# Autodesk Inventor assembly: drivebay
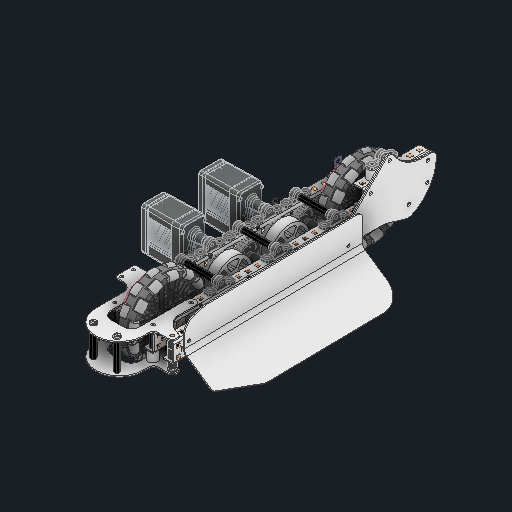
[picture p0: Inventor's stored thumbnail of the model, 512x512]
Saved by Autodesk Inventor 2024 (Build 280153000, 153)
## iProperties
Created: 2023-08-15
Part Number: drivebay
Document SubType Name: Assembly
Designer: avere
Author: avere
## Documents named in this file (25)
- D:\vex_robotics\hardware\cad\spades_v0.1\chassis\drivebay.iam
- D:\vex_robotics\hardware\cad\spades_v0.1\chassis\outer.iam
- D:\vex_robotics\hardware\cad\spades_v0.1\chassis\inner.iam
- D:\vex_robotics\hardware\cad\spades_v0.1\chassis\wheel.iam
- D:\vex_robotics\hardware\cad\spades_v0.1\chassis\gear.iam
- D:\vex_robotics\hardware\cad\VEX-CAD-Inventor-1.41\Motion\Spacers\Spacer Nylon .500 OD\NSpacer White .500 OD x .500.ipt
- D:\vex_robotics\hardware\cad\spades_v0.1\chassis\custom_parts\gusset.ipt
- D:\vex_robotics\hardware\cad\VEX-CAD-Inventor-1.41\Structure\Standoff\Standoff 1.50.ipt
- D:\vex_robotics\hardware\cad\VEX-CAD-Inventor-1.41\Motion\Spacers\Spacer Nylon .375 OD\NSpacer .375 OD x .125.ipt
- D:\vex_robotics\hardware\cad\spades_v0.1\chassis\flapper.iam
- D:\vex_robotics\hardware\cad\VEX-CAD-Inventor-1.41\Motion\Spacers\Spacer Nylon .375 OD\NSpacer .375 OD x .375.ipt
- D:\vex_robotics\hardware\cad\VEX-CAD-Inventor-1.41\Motion\Spacers\Washer Steel\SWasher .375 OD x .062500.ipt
- D:\vex_robotics\hardware\cad\VEX-CAD-Inventor-1.41\Motion\Spacers\Washer Steel\SWasher .375 OD x .015625.ipt
- D:\vex_robotics\hardware\cad\VEX-CAD-Inventor-1.41\Motion\Spacers\Washer Teflon\TWasher .375 OD x .04000.ipt
- D:\vex_robotics\hardware\cad\spades_v0.1\chassis\flex_wheel.iam
- D:\vex_robotics\hardware\cad\VEX-CAD-Inventor-1.41\Structure\C Channel\Aluminum 1x2x1\Alu C 1x2x1x7.ipt
- D:\vex_robotics\hardware\cad\VEX-CAD-Inventor-1.41\Motion\Shaft LS\LS Pillow Bearing Block.ipt
- D:\vex_robotics\hardware\cad\spades_v0.1\chassis\custom_parts\sled.ipt
- D:\vex_robotics\hardware\cad\hardware\Nylon Screw Pan-Head .375.ipt
- D:\vex_robotics\hardware\cad\VEX-CAD-Inventor-1.41\Motion\Spacers\Spacer Nylon .500 OD.ipt
- D:\vex_robotics\hardware\cad\VEX-CAD-Inventor-1.41\Structure\Standoff.ipt
- D:\vex_robotics\hardware\cad\VEX-CAD-Inventor-1.41\Motion\Spacers\Spacer Nylon .375 OD.ipt
- D:\vex_robotics\hardware\cad\VEX-CAD-Inventor-1.41\Motion\Spacers\Washer Steel.ipt
- D:\vex_robotics\hardware\cad\VEX-CAD-Inventor-1.41\Motion\Spacers\Washer Teflon.ipt
- D:\vex_robotics\hardware\cad\VEX-CAD-Inventor-1.41\Motion\Shaft LS\Shaft Collar ipts\Shaft Collar Set Screw.ipt
## Components (44 placed, 19 different names)
1. outer:1 [sub-assembly] — Insert:3, Insert:4, Insert:27, Insert:29, Insert:31, Insert:32, Insert:39, Insert:40, Insert:41, Mate:5, Mate:8, Mate:10, Mate:11
2. inner:1 [sub-assembly] — Insert:10, Mate:3, Insert:11, Mate:4, Insert:12, Mate:9, Insert:49, Insert:50, Insert:55
3. wheel:1 [sub-assembly] — Insert:3
4. wheel:2 [sub-assembly] — Insert:4
5. gear:1 [sub-assembly] — Insert:31
6. gear:2 [sub-assembly] — Insert:27
7. gear:5 [sub-assembly] — Insert:29
8. gusset:1 — Insert:10, Mate:3, Insert:16, Insert:17, Insert:34, Insert:51, Insert:52
9. gusset:2 — Insert:11, Mate:4, Insert:13, Insert:14, Insert:15, Insert:53, Insert:54
10. NSpacer White .500 OD x .500:1 — Insert:12
11. NSpacer White .500 OD x .500:2 — Insert:13
12. NSpacer White .500 OD x .500:3 — Insert:14
13. NSpacer White .500 OD x .500:4 — Insert:15
14. Standoff 1.50:1 — Insert:17
15. Standoff 1.50:2 — Insert:16
16. Standoff 1.50:3 — Insert:18, Insert:19
17. NSpacer .375 OD x .125:1 — Insert:18, Mate:11
18. NSpacer .375 OD x .125:2 — Insert:19, Insert:50
19. Standoff 1.50:4
20. NSpacer .375 OD x .125:3 — Mate:9
21. NSpacer .375 OD x .125:4 — Insert:32
22. Standoff 1.50:5
23. NSpacer .375 OD x .125:5 — Mate:10
24. NSpacer .375 OD x .125:6 — Insert:49
25. flapper:2 [sub-assembly] — Insert:34, Insert:38
26. NSpacer .375 OD x .375:7 — Insert:37, Insert:38
27. SWasher .375 OD x .062500:1 — Insert:35, Insert:37
28. SWasher .375 OD x .015625:2 — Insert:36
29. TWasher .375 OD x .04000:1 — Insert:35, Insert:36
30. flex_wheel:1 [sub-assembly] — Insert:39
31. flex_wheel:2 [sub-assembly] — Insert:40
32. Alu C 1x2x1x7:1 — Insert:41, Mate:5, Insert:45, Insert:48
33. LS Pillow Bearing Block:1 — Insert:47
34. NSpacer White .500 OD x .500:5
35. NSpacer White .500 OD x .500:6 — Insert:48
36. NSpacer .375 OD x .125:8 — Insert:47
37. SWasher .375 OD x .062500:3 — Insert:46
38. sled:1 — Insert:44, Mate:7
39. sled:2 — Insert:44, Mate:7, Insert:45, Mate:8, Insert:46
40. Nylon Screw Pan-Head .375:1 — Insert:52
41. Nylon Screw Pan-Head .375:2 — Insert:51
42. Nylon Screw Pan-Head .375:3 — Insert:54
43. Nylon Screw Pan-Head .375:4 — Insert:53
44. Shaft Collar Set Screw:1 — Insert:55
## Relationships (51: Insert 42, Mate 9)
- Insert:3 (13.716 mm): outer:1 ↔ wheel:1
- Insert:4 (13.716 mm): outer:1 ↔ wheel:2
- Insert:10: inner:1 ↔ gusset:1
- Mate:3: inner:1 ↔ gusset:1
- Insert:11 (12.7 mm): inner:1 ↔ gusset:2
- Mate:4: inner:1 ↔ gusset:2
- Insert:12: inner:1 ↔ NSpacer White .500 OD x .500:1
- Insert:13: gusset:2 ↔ NSpacer White .500 OD x .500:2
- Insert:14: gusset:2 ↔ NSpacer White .500 OD x .500:3
- Insert:15: gusset:2 ↔ NSpacer White .500 OD x .500:4
- Insert:16: gusset:1 ↔ Standoff 1.50:2
- Insert:17: gusset:1 ↔ Standoff 1.50:1
- Insert:18: Standoff 1.50:3 ↔ NSpacer .375 OD x .125:1
- Insert:19: Standoff 1.50:3 ↔ NSpacer .375 OD x .125:2
- [Insert]: Standoff 1.50:4 ↔ NSpacer .375 OD x .125:3
- [Insert]: Standoff 1.50:4 ↔ NSpacer .375 OD x .125:4
- [Insert]: Standoff 1.50:5 ↔ NSpacer .375 OD x .125:5
- [Insert]: Standoff 1.50:5 ↔ NSpacer .375 OD x .125:6
- Insert:27 (1.27 mm): outer:1 ↔ gear:2
- Insert:29 (1.27 mm): outer:1 ↔ gear:5
- Insert:31 (1.27 mm): outer:1 ↔ gear:1
- Insert:32: outer:1 ↔ NSpacer .375 OD x .125:4
- Insert:34: gusset:1 ↔ flapper:2
- Insert:35: SWasher .375 OD x .062500:1 ↔ TWasher .375 OD x .04000:1
- Insert:36: SWasher .375 OD x .015625:2 ↔ TWasher .375 OD x .04000:1
- Insert:37: NSpacer .375 OD x .375:7 ↔ SWasher .375 OD x .062500:1
- Insert:38: flapper:2 ↔ NSpacer .375 OD x .375:7
- Insert:39 (1.27 mm): outer:1 ↔ flex_wheel:1
- Insert:40 (1.27 mm): outer:1 ↔ flex_wheel:2
- Insert:41: outer:1 ↔ Alu C 1x2x1x7:1
- Mate:5: outer:1 ↔ Alu C 1x2x1x7:1
- [Insert]: LS Pillow Bearing Block:1 ↔ NSpacer White .500 OD x .500:5
- [Mate]: LS Pillow Bearing Block:1 ↔ NSpacer White .500 OD x .500:6
- [Insert]: NSpacer .375 OD x .125:8 ↔ SWasher .375 OD x .062500:3
- Insert:44: sled:1 ↔ sled:2
- Mate:7: sled:1 ↔ sled:2
- Insert:45: Alu C 1x2x1x7:1 ↔ sled:2
- Mate:8: outer:1 ↔ sled:2
- Insert:46: SWasher .375 OD x .062500:3 ↔ sled:2
- Insert:47: LS Pillow Bearing Block:1 ↔ NSpacer .375 OD x .125:8
- Insert:48: Alu C 1x2x1x7:1 ↔ NSpacer White .500 OD x .500:6
- Mate:9: inner:1 ↔ NSpacer .375 OD x .125:3
- Insert:49: inner:1 ↔ NSpacer .375 OD x .125:6
- Mate:10: outer:1 ↔ NSpacer .375 OD x .125:5
- Insert:50: inner:1 ↔ NSpacer .375 OD x .125:2
- Mate:11: outer:1 ↔ NSpacer .375 OD x .125:1
- Insert:51: gusset:1 ↔ Nylon Screw Pan-Head .375:2
- Insert:52: gusset:1 ↔ Nylon Screw Pan-Head .375:1
- Insert:53: gusset:2 ↔ Nylon Screw Pan-Head .375:4
- Insert:54: gusset:2 ↔ Nylon Screw Pan-Head .375:3
- Insert:55: inner:1 ↔ Shaft Collar Set Screw:1
## Named parameters: d70_d67 = 0 mm, d71_d68 = 0 mm, d73_d67 = 0 mm, d74_d68 = 0 mm
